# Autodesk Inventor assembly: Intake motor + pulley & wheel on xrail left
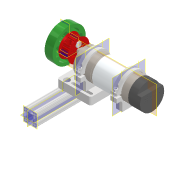
[picture p0: Inventor's stored thumbnail of the model, 180x180]
Saved by Autodesk Inventor 2020 (Build 240168000, 168)
## iProperties
Created: 2020-01-13
Part Number: Intake motor + pulley & wheel on xrail left
Document SubType Name: Assembly
Designer: ball
Author: ball
## Documents named in this file (4)
- C:\FTC\FTC8863CAD\2019 Robot\Collection\Intake\Intake motor + pulley & wheel on xrail left.iam
- C:\FTC\FTC8863CAD\Actobotics\565 parts\xrail_3.5in.ipt
- C:\FTC\FTC8863CAD\2019 Robot\Collection\intake motor mount to xrail.ipt
- C:\FTC\FTC8863CAD\2019 Robot\Collection\Intake\Intake motor + pulley & 2 inch compliant wheel left.iam
## Components (3 placed, 3 different names)
1. Intake motor + pulley & 2 inch compliant wheel left:1 [sub-assembly]
2. xrail_3.5in:1 — Flush:4
3. intake motor mount to xrail:1 — Flush:4
## Relationships (6: Flush 4, Mate 2)
- [Mate]: xrail_3.5in:1 ↔ intake motor mount to xrail:1
- [Flush]: xrail_3.5in:1 ↔ intake motor mount to xrail:1
- [Mate]: Intake motor + pulley & 2 inch compliant wheel left:1 ↔ intake motor mount to xrail:1
- [Flush] (5.08 mm): Intake motor + pulley & 2 inch compliant wheel left:1 ↔ intake motor mount to xrail:1
- Flush:4: xrail_3.5in:1 ↔ intake motor mount to xrail:1
- [Flush] (2.3114 mm): Intake motor + pulley & 2 inch compliant wheel left:1 ↔ intake motor mount to xrail:1
